# Autodesk Inventor assembly: Assembly8
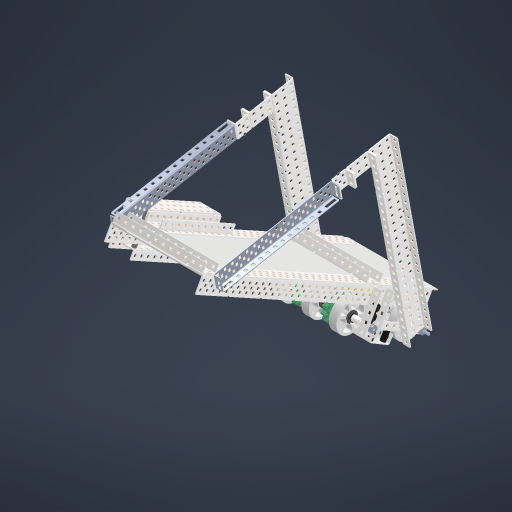
[picture p0: Inventor's stored thumbnail of the model, 512x512]
Saved by Autodesk Inventor 2023 (Build 270158000, 158)
## iProperties
Created: 2023-02-05
Part Number: Assembly8
Document SubType Name: Assembly
Designer: Windows Macbook
Author: Windows Macbook
## Documents named in this file (34)
- C:\Users\Windows Macbook\Desktop\Inventor\Assembly8.iam
- C:\Users\Windows Macbook\Documents\Inventor\Content Center Files\VEX-CAD-Inventor-1.4.0\Structure\Angle\Aluminum\2x2\Alu Angle 2x2x35.ipt
- C:\Users\Windows Macbook\Documents\Inventor\Content Center Files\VEX-CAD-Inventor-1.4.0\Motion\Spacers\Spacer Nylon .313 OD\NSpacer .313 OD x .125.ipt
- C:\Users\Windows Macbook\Documents\Inventor\Content Center Files\VEX-CAD-Inventor-1.4.0\Motion\Spacers\Spacer Nylon .313 OD.ipt
- C:\Users\Windows Macbook\Documents\Inventor\Content Center Files\VEX-CAD-Inventor-1.4.0\Structure\C Channel\Aluminum 1x3x1\Alu C 1x3x1x2.ipt
- C:\Users\Windows Macbook\Documents\Inventor\Content Center Files\VEX-CAD-Inventor-1.4.0\Structure\C Channel\Aluminum 1x2x1\Alu C 1x2x1x2.ipt
- C:\Users\Windows Macbook\Documents\Inventor\Content Center Files\VEX-CAD-Inventor-1.4.0\Structure\Chassis Rails\Steel Chassis Rail 2x1x16.ipt
- C:\Users\Windows Macbook\Documents\Inventor\Content Center Files\VEX-CAD-Inventor-1.4.0\Structure\C Channel\Aluminum 1x3x1\Alu C 1x3x1x25.ipt
- C:\Users\Windows Macbook\Documents\Inventor\Content Center Files\VEX-CAD-Inventor-1.4.0\Structure\C Channel\Aluminum 1x2x1\Alu C 1x2x1x12.ipt
- C:\Users\Windows Macbook\Desktop\Inventor\abs.ipt
- C:\Users\Windows Macbook\Documents\Inventor\Content Center Files\VEX-CAD-Inventor-1.4.0\Motion\Wheels\Flex Wheels\4.000 Flex Wheel\4.000 30A 1.000.ipt
- C:\Users\Windows Macbook\Documents\Inventor\Content Center Files\VEX-CAD-Inventor-1.4.0\Motion\Wheels\Flex Wheels\4.000 Flex Wheel.ipt
- C:\Users\Windows Macbook\Documents\Inventor\Content Center Files\VEX-CAD-Inventor-1.4.0\Motion\Wheels\Flex Wheels\VersaHub.ipt
- C:\Users\Windows Macbook\Documents\Inventor\Content Center Files\VEX-CAD-Inventor-1.4.0\Motion\Wheels\Flex Wheels\VersaHex Adapters .250.ipt
- C:\Users\Windows Macbook\Documents\Inventor\Content Center Files\276-7500-001 Web.ipt
- C:\Users\Windows Macbook\Documents\Inventor\Content Center Files\VEX-CAD-Inventor-1.4.0\Motion\Spacers\Spacer Nylon .313 OD\NSpacer .313 OD x .500.ipt
- C:\Users\Windows Macbook\Documents\Inventor\Content Center Files\VEX-CAD-Inventor-1.4.0\Structure\C Channel\Aluminum 1x3x1\Alu C 1x3x1x11.ipt
- C:\Users\Windows Macbook\Documents\Inventor\Content Center Files\VEX-CAD-Inventor-1.4.0\Structure\Standoff\Standoff 2.00.ipt
- C:\Users\Windows Macbook\Documents\Inventor\Content Center Files\VEX-CAD-Inventor-1.4.0\Structure\Standoff.ipt
- C:\Users\Windows Macbook\Documents\Inventor\Content Center Files\VEX-CAD-Inventor-1.4.0\Motion\Insert Square.ipt
- C:\Users\Windows Macbook\Documents\Inventor\Content Center Files\VEX-CAD-Inventor-1.4.0\Structure\C Channel\Aluminum 1x2x1\Alu C 1x2x1x11.ipt
- C:\Users\Windows Macbook\Documents\Inventor\Content Center Files\VEX-CAD-Inventor-1.4.0\Structure\C Channel\Aluminum 1x2x1\Alu C 1x2x1x5.ipt
- C:\Users\Windows Macbook\Documents\Inventor\Content Center Files\VEX-CAD-Inventor-1.4.0\Motion\Shaft LS\Bearing Flat.ipt
- C:\Users\Windows Macbook\Documents\Inventor\Content Center Files\VEX-CAD-Inventor-1.4.0\Motion\Shaft LS\Shaft LS.ipt
- C:\Users\Windows Macbook\Documents\Inventor\Content Center Files\VEX-CAD-Inventor-1.4.0\Motion\Shaft LS\Shaft Collar Metal.ipt
- C:\Users\Windows Macbook\Documents\Inventor\Content Center Files\VEX-CAD-Inventor-1.4.0\Motion\Shaft LS\Shaft LS\Shaft LS 7.5.ipt
- C:\Users\Windows Macbook\Documents\Inventor\Content Center Files\VEX-CAD-Inventor-1.4.0\Motion\Shaft LS\Shaft LS\Shaft LS 6.5.ipt
- C:\Users\Windows Macbook\Documents\Inventor\Content Center Files\flex2.iam
- C:\Users\Windows Macbook\Documents\Inventor\Content Center Files\VEX-CAD-Inventor-1.4.0\Structure\Angle\Aluminum\1x1\Alu Angle 1x1x10.ipt
- C:\Users\Windows Macbook\Documents\Inventor\Content Center Files\VEX-CAD-Inventor-1.4.0\Motion\Spacers\Spacer Nylon .313 OD\NSpacer .313 OD x .250.ipt
- C:\Users\Windows Macbook\Documents\Inventor\Content Center Files\VEX-CAD-Inventor-1.4.0\Motion\Spacers\Spacer Plastic\PSpacer 8.0.ipt
- C:\Users\Windows Macbook\Documents\Inventor\Content Center Files\VEX-CAD-Inventor-1.4.0\Motion\Spacers\Spacer Plastic.ipt
- C:\Users\Windows Macbook\Documents\Inventor\Content Center Files\VEX-CAD-Inventor-1.4.0\Motion\Sprockets\9P Sprocket\9P 12T Sprocket, Square.iam
- C:\Users\Windows Macbook\Documents\Inventor\Content Center Files\VEX-CAD-Inventor-1.4.0\Motion\Sprockets\9P Sprocket.iam
## Components (69 placed, 27 different names)
1. Alu Angle 2x2x35:2 — Insert:21, Angle:2, Insert:23, Mate:5, Mate:6, Flush:11, Insert:69, Insert:70, Insert:87, Insert:88
2. Alu C 1x3x1x25:1 — Mate:4, Flush:9, Flush:10, Insert:22, Flush:13
3. NSpacer .313 OD x .125:1 — Insert:21, Insert:22
4. NSpacer .313 OD x .125:2 — Insert:23
5. Alu C 1x3x1x2:1 — Insert:19, Insert:20, Mate:4, Flush:9, Flush:10
6. Alu C 1x2x1x2:1 — Insert:19, Insert:20, Mate:3, Flush:7, Flush:8
7. Steel Chassis Rail 2x1x16:1 — Mate:3, Flush:7, Flush:8, Angle:2
8. Alu C 1x2x1x12:3 — Insert:69, Insert:70
9. abs:1 — Mate:5, Mate:6, Flush:11, Mate:7, Mate:8, Flush:12, Mate:16
10. Alu Angle 2x2x35:3 — Mate:7, Mate:8, Flush:12, Insert:30, Insert:36, Insert:81, Insert:82, Insert:83, Insert:84, Insert:89, Insert:90
11. NSpacer .313 OD x .125:3 — Insert:30, Insert:31
12. Alu C 1x3x1x25:2 — Insert:31, Flush:13, Insert:34, Insert:35
13. Alu C 1x3x1x2:2 — Insert:34, Insert:35
14. Alu C 1x2x1x2:2 — Flush:14, Flush:15, Mate:9, Mate:21, Flush:16, Flush:17
15. Steel Chassis Rail 2x1x16:2 — Flush:14, Flush:15, Mate:9
16. NSpacer .313 OD x .125:4 — Insert:36
17. 4.000 30A 1.000:1
18. VersaHub:1
19. VersaHub:2 — Mate:18, Mate:19, Mate:20
20. VersaHex Adapters .250:2 — Insert:59
21. 276-7500-001 Web:1 — Mate:16
22. Alu C 1x3x1x11:3 — Insert:80
23. NSpacer .313 OD x .500:5 — Insert:60
24. Alu C 1x2x1x11:1 — Insert:80, Insert:81, Insert:82
25. Alu C 1x3x1x11:2 — Insert:52, Insert:53
26. Standoff 2.00:1 — Insert:53
27. Standoff 2.00:2 — Insert:52
28. Standoff 2.00:3
29. Standoff 2.00:4
30. Insert Square:1 — Insert:59, Insert:60
31. VersaHex Adapters .250:3 — Mate:18, Mate:19, Mate:20
32. Insert Square:2
33. Steel Chassis Rail 2x1x16:3 — Mate:21, Flush:16, Flush:17
34. Alu C 1x2x1x12:4 — Insert:83, Insert:84
35. Alu C 1x2x1x5:2 — Insert:89, Insert:90, Insert:93, Insert:94
36. Alu C 1x2x1x5:1 — Insert:87, Insert:88, Insert:95, Insert:96
37. NSpacer .313 OD x .250:6 — Insert:99
38. NSpacer .313 OD x .250:7 — Insert:100
39. Bearing Flat:1 — Insert:93, Insert:94, Insert:97
40. Bearing Flat:2 — Insert:95, Insert:96, Insert:98
41. Shaft LS 7.5:1 — Flush:18, Rigid:1
42. Shaft Collar Metal:1 — Insert:97
43. Shaft Collar Metal:2 — Insert:98, Flush:18, Rigid:1
44. Alu Angle 1x1x10:1 — Insert:99, Flush:19, Insert:101, Insert:106, Insert:108, Insert:109, Insert:121
45. Alu Angle 1x1x10:2 — Flush:19, Insert:100, Insert:102, Insert:104, Insert:110, Insert:111, Insert:122
46. Shaft Collar Metal:3 — Insert:101, Flush:20, Cylindrical:1
47. Shaft Collar Metal:4 — Insert:102
48. Shaft LS 6.5:2 — Flush:20, Cylindrical:1
49. flex2:1 [sub-assembly] — Insert:103
50. flex2:2 [sub-assembly] — Insert:107
51. NSpacer .313 OD x .500:8 — Insert:103, Insert:104
52. flex2:3 [sub-assembly] — Insert:107
53. NSpacer .313 OD x .500:9 — Insert:106
54. PSpacer 8.0:1 — Insert:109, Insert:113
55. PSpacer 8.0:2 — Insert:108, Insert:112
56. PSpacer 8.0:3 — Insert:111, Insert:114
57. PSpacer 8.0:4 — Insert:110, Insert:115
58. Alu C 1x3x1x11:4 — Insert:116, Insert:117
59. PSpacer 8.0:5 — Insert:112
60. PSpacer 8.0:6 — Insert:113
61. PSpacer 8.0:7 — Insert:114, Insert:117
62. PSpacer 8.0:8 — Insert:115, Insert:116
63. flex2:4 [sub-assembly] — Insert:123
64. flex2:5 [sub-assembly] — Insert:125
65. NSpacer .313 OD x .500:10 — Insert:122
66. flex2:6 [sub-assembly] — Insert:124
67. NSpacer .313 OD x .500:11 — Insert:121
68. 9P 12T Sprocket, Square:1 [sub-assembly] — Insert:124, Insert:125
69. 9P 12T Sprocket, Square:2 [sub-assembly] — Insert:123
## Relationships (104: Insert 72, Mate 15, Flush 14, Angle 1, WeldJoint 1, CylindricalJoint 1)
- Insert:19: Alu C 1x3x1x2:1 ↔ Alu C 1x2x1x2:1
- Insert:20: Alu C 1x3x1x2:1 ↔ Alu C 1x2x1x2:1
- Mate:3: Alu C 1x2x1x2:1 ↔ Steel Chassis Rail 2x1x16:1
- Flush:7: Alu C 1x2x1x2:1 ↔ Steel Chassis Rail 2x1x16:1
- Flush:8: Alu C 1x2x1x2:1 ↔ Steel Chassis Rail 2x1x16:1
- Mate:4: Alu C 1x3x1x25:1 ↔ Alu C 1x3x1x2:1
- Flush:9: Alu C 1x3x1x25:1 ↔ Alu C 1x3x1x2:1
- Flush:10: Alu C 1x3x1x25:1 ↔ Alu C 1x3x1x2:1
- Insert:21: Alu Angle 2x2x35:2 ↔ NSpacer .313 OD x .125:1
- Insert:22: Alu C 1x3x1x25:1 ↔ NSpacer .313 OD x .125:1
- Angle:2 (50.5 deg): Alu Angle 2x2x35:2 ↔ Steel Chassis Rail 2x1x16:1
- Insert:23: Alu Angle 2x2x35:2 ↔ NSpacer .313 OD x .125:2
- Mate:5: Alu Angle 2x2x35:2 ↔ abs:1
- Mate:6: Alu Angle 2x2x35:2 ↔ abs:1
- Flush:11 (12.7 mm): Alu Angle 2x2x35:2 ↔ abs:1
- Mate:7: abs:1 ↔ Alu Angle 2x2x35:3
- Mate:8: abs:1 ↔ Alu Angle 2x2x35:3
- Flush:12 (12.7 mm): abs:1 ↔ Alu Angle 2x2x35:3
- Insert:30: Alu Angle 2x2x35:3 ↔ NSpacer .313 OD x .125:3
- Insert:31: NSpacer .313 OD x .125:3 ↔ Alu C 1x3x1x25:2
- Flush:13: Alu C 1x3x1x25:1 ↔ Alu C 1x3x1x25:2
- [Insert]: Alu C 1x3x1x2:2 ↔ Alu C 1x2x1x2:2
- [Insert]: Alu C 1x3x1x2:2 ↔ Alu C 1x2x1x2:2
- Insert:34: Alu C 1x3x1x25:2 ↔ Alu C 1x3x1x2:2
- Insert:35: Alu C 1x3x1x25:2 ↔ Alu C 1x3x1x2:2
- Flush:14: Alu C 1x2x1x2:2 ↔ Steel Chassis Rail 2x1x16:2
- Flush:15: Alu C 1x2x1x2:2 ↔ Steel Chassis Rail 2x1x16:2
- Mate:9: Alu C 1x2x1x2:2 ↔ Steel Chassis Rail 2x1x16:2
- Insert:36: Alu Angle 2x2x35:3 ↔ NSpacer .313 OD x .125:4
- [Insert]: 4.000 30A 1.000:1 ↔ VersaHub:2
- [Insert]: 4.000 30A 1.000:1 ↔ VersaHub:2
- [Insert]: 4.000 30A 1.000:1 ↔ VersaHub:1
- [Insert]: 4.000 30A 1.000:1 ↔ VersaHub:1
- [Mate]: VersaHub:1 ↔ VersaHex Adapters .250:2
- [Mate]: VersaHub:1 ↔ VersaHex Adapters .250:2
- [Mate]: VersaHub:1 ↔ VersaHex Adapters .250:2
- Mate:16: abs:1 ↔ 276-7500-001 Web:1
- [Insert]: Alu C 1x3x1x11:3 ↔ NSpacer .313 OD x .500:5
- [Insert]: Alu C 1x3x1x11:3 ↔ Standoff 2.00:1
- [Insert]: Alu C 1x3x1x11:3 ↔ Standoff 2.00:3
- [Insert]: Alu C 1x3x1x11:3 ↔ Standoff 2.00:4
- [Insert]: Alu C 1x3x1x11:3 ↔ Standoff 2.00:2
- Insert:52: Alu C 1x3x1x11:2 ↔ Standoff 2.00:2
- Insert:53: Alu C 1x3x1x11:2 ↔ Standoff 2.00:1
- Insert:59: VersaHex Adapters .250:2 ↔ Insert Square:1
- Insert:60: NSpacer .313 OD x .500:5 ↔ Insert Square:1
- Insert:69: Alu Angle 2x2x35:2 ↔ Alu C 1x2x1x12:3
- Insert:70: Alu Angle 2x2x35:2 ↔ Alu C 1x2x1x12:3
- [Insert]: Alu C 1x3x1x11:3 ↔ Alu C 1x2x1x11:1
- [Insert]: VersaHex Adapters .250:3 ↔ Insert Square:2
- Mate:18: VersaHub:2 ↔ VersaHex Adapters .250:3
- Mate:19: VersaHub:2 ↔ VersaHex Adapters .250:3
- Mate:20: VersaHub:2 ↔ VersaHex Adapters .250:3
- Insert:80: Alu C 1x3x1x11:3 ↔ Alu C 1x2x1x11:1
- Mate:21: Alu C 1x2x1x2:2 ↔ Steel Chassis Rail 2x1x16:3
- Flush:16: Alu C 1x2x1x2:2 ↔ Steel Chassis Rail 2x1x16:3
- Flush:17: Alu C 1x2x1x2:2 ↔ Steel Chassis Rail 2x1x16:3
- Insert:81: Alu Angle 2x2x35:3 ↔ Alu C 1x2x1x11:1
- Insert:82: Alu Angle 2x2x35:3 ↔ Alu C 1x2x1x11:1
- Insert:83: Alu Angle 2x2x35:3 ↔ Alu C 1x2x1x12:4
- Insert:84: Alu Angle 2x2x35:3 ↔ Alu C 1x2x1x12:4
- Insert:87: Alu Angle 2x2x35:2 ↔ Alu C 1x2x1x5:1
- Insert:88: Alu Angle 2x2x35:2 ↔ Alu C 1x2x1x5:1
- Insert:89: Alu Angle 2x2x35:3 ↔ Alu C 1x2x1x5:2
- Insert:90: Alu Angle 2x2x35:3 ↔ Alu C 1x2x1x5:2
- [Insert]: Alu C 1x2x1x5:2 ↔ NSpacer .313 OD x .250:6
- [Insert]: Alu C 1x2x1x5:1 ↔ NSpacer .313 OD x .250:7
- Insert:93: Alu C 1x2x1x5:2 ↔ Bearing Flat:1
- Insert:94: Alu C 1x2x1x5:2 ↔ Bearing Flat:1
- Insert:95: Alu C 1x2x1x5:1 ↔ Bearing Flat:2
- Insert:96: Alu C 1x2x1x5:1 ↔ Bearing Flat:2
- Insert:97: Bearing Flat:1 ↔ Shaft Collar Metal:1
- Insert:98: Bearing Flat:2 ↔ Shaft Collar Metal:2
- Flush:18: Shaft LS 7.5:1 ↔ Shaft Collar Metal:2
- Rigid:1 [WeldJoint]: Shaft LS 7.5:1 ↔ Shaft Collar Metal:2
- Insert:99: NSpacer .313 OD x .250:6 ↔ Alu Angle 1x1x10:1
- Flush:19: Alu Angle 1x1x10:1 ↔ Alu Angle 1x1x10:2
- Insert:100: NSpacer .313 OD x .250:7 ↔ Alu Angle 1x1x10:2
- Insert:101: Alu Angle 1x1x10:1 ↔ Shaft Collar Metal:3
- Insert:102: Alu Angle 1x1x10:2 ↔ Shaft Collar Metal:4
- Flush:20: Shaft Collar Metal:3 ↔ Shaft LS 6.5:2
- Cylindrical:1: Shaft Collar Metal:3 ↔ Shaft LS 6.5:2
- Insert:103: flex2:1 ↔ NSpacer .313 OD x .500:8
- Insert:104: Alu Angle 1x1x10:2 ↔ NSpacer .313 OD x .500:8
- [Insert]: flex2:3 ↔ NSpacer .313 OD x .500:9
- Insert:106: Alu Angle 1x1x10:1 ↔ NSpacer .313 OD x .500:9
- Insert:107 (30.7518 mm): flex2:2 ↔ flex2:3
- Insert:108: Alu Angle 1x1x10:1 ↔ PSpacer 8.0:2
- Insert:109: Alu Angle 1x1x10:1 ↔ PSpacer 8.0:1
- Insert:110: Alu Angle 1x1x10:2 ↔ PSpacer 8.0:4
- Insert:111: Alu Angle 1x1x10:2 ↔ PSpacer 8.0:3
- Insert:112: PSpacer 8.0:2 ↔ PSpacer 8.0:5
- Insert:113: PSpacer 8.0:1 ↔ PSpacer 8.0:6
- Insert:114: PSpacer 8.0:3 ↔ PSpacer 8.0:7
- Insert:115: PSpacer 8.0:4 ↔ PSpacer 8.0:8
- Insert:116: Alu C 1x3x1x11:4 ↔ PSpacer 8.0:8
- Insert:117: Alu C 1x3x1x11:4 ↔ PSpacer 8.0:7
- [Insert]: flex2:4 ↔ NSpacer .313 OD x .500:10
- [Insert]: flex2:6 ↔ NSpacer .313 OD x .500:11
- Insert:121: Alu Angle 1x1x10:1 ↔ NSpacer .313 OD x .500:11
- Insert:122: Alu Angle 1x1x10:2 ↔ NSpacer .313 OD x .500:10
- Insert:123 (5.08 mm): flex2:4 ↔ 9P 12T Sprocket, Square:2
- Insert:124 (5.08 mm): flex2:6 ↔ 9P 12T Sprocket, Square:1
- Insert:125 (9.525 mm): flex2:5 ↔ 9P 12T Sprocket, Square:1
## Named parameters: d66_d36 = 0 mm, d67_d37 = 0 mm, d74_d58 = 0 mm, d75_d59 = 0 mm, d76_d50 = 0 mm, d77_d51 = 0 mm, d79_d53 = 0 mm, d83_d57 = 0 mm, d124_d107 = 0 mm, d171_d169 = 0 mm, d186_d169 = 0 mm, d187_d171_d169 = 0 mm
